# Autodesk Inventor assembly: 5DržačaLidara
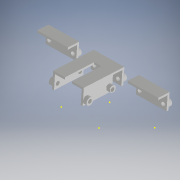
[picture p0: Inventor's stored thumbnail of the model, 180x180]
Saved by Autodesk Inventor 2020 (Build 240168000, 168)
## iProperties
Created: 2020-07-11
Part Number: 5DržačaLidara
Document SubType Name: Assembly
Designer: Sičaja
Author: Sičaja
## Documents named in this file (2)
- C:\Users\Sicaja\Desktop\Draws_Inventor\Inventor_Robocup\5DržačaLidara.iam
- C:\Users\Sicaja\Desktop\Draws_Inventor\Inventor_Robocup\DržačSenzoraUdaljenostiOnlyOne(1)_v.1.0.ipt
## Components (5 placed, 1 different names)
1. DržačSenzoraUdaljenostiOnlyOne(1)_v.1.0:2 — Mate:1, Mate:5
2. DržačSenzoraUdaljenostiOnlyOne(1)_v.1.0:3 — Mate:3, Mate:4
3. DržačSenzoraUdaljenostiOnlyOne(1)_v.1.0:1
4. DržačSenzoraUdaljenostiOnlyOne(1)_v.1.0:4 — Mate:1, Mate:3, Mate:4, Mate:5
5. DržačSenzoraUdaljenostiOnlyOne(1)_v.1.0:5
## Component patterns: (3 elements, first: DržačSenzoraUdaljenostiOnlyOne(1)_v.1.0:1)
## Relationships (4: Mate 4)
- Mate:1: DržačSenzoraUdaljenostiOnlyOne(1)_v.1.0:2 ↔ DržačSenzoraUdaljenostiOnlyOne(1)_v.1.0:4
- Mate:3: DržačSenzoraUdaljenostiOnlyOne(1)_v.1.0:3 ↔ DržačSenzoraUdaljenostiOnlyOne(1)_v.1.0:4
- Mate:4: DržačSenzoraUdaljenostiOnlyOne(1)_v.1.0:3 ↔ DržačSenzoraUdaljenostiOnlyOne(1)_v.1.0:4
- Mate:5: DržačSenzoraUdaljenostiOnlyOne(1)_v.1.0:2 ↔ DržačSenzoraUdaljenostiOnlyOne(1)_v.1.0:4
